# Autodesk Inventor assembly: StraightMF_DSS
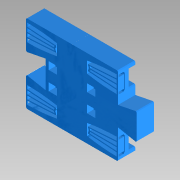
[picture p0: Inventor's stored thumbnail of the model, 180x180]
Saved by Autodesk Inventor 2021 (Build 250183000, 183)
## iProperties
Created: 2021-03-01
Part Number: StraightMF_DSS
Document SubType Name: Assembly
Designer: kumagai
Author: kumagai
## Documents named in this file (11)
- X:\Develop\CAD\PlaRails\StraightRail\StraightRail_i.iam
- X:\Develop\CAD\PlaRails\RailJointMale.ipt
- X:\Develop\CAD\PlaRails\RailJointFemale.ipt
- X:\Develop\CAD\PlaRails\GlobalParameter.ipt
- StraightFF26.iam
- StraightFF60.iam
- StraightMF134.iam
- StraightMF215.iam
- StraightMF_DSS.iam
- StraightMM26.iam
- StraightMM60.iam
## Components (4 placed, 4 different names)
1. M1 — フラッシュ:1, フラッシュ:3, フラッシュ:4
2. M2 — フラッシュ:2, メイト:1, メイト:2
3. F1 — フラッシュ:5, メイト:3, メイト:4
4. F2 — フラッシュ:6, フラッシュ:7, フラッシュ:8
## Relationships (12: Flush 8, Mate 4)
- フラッシュ:1 [Flush]: M1
- フラッシュ:2 [Flush]: M2
- フラッシュ:3 [Flush] (-7.264 mm): M1
- メイト:1 [Mate]: M2
- フラッシュ:4 [Flush]: M1
- メイト:2 [Mate]: M2
- フラッシュ:5 [Flush]: F1
- フラッシュ:6 [Flush]: F2
- フラッシュ:7 [Flush] (-7.264 mm): F2
- フラッシュ:8 [Flush]: F2
- メイト:3 [Mate]: F1
- メイト:4 [Mate]: F1
## Named parameters: Length = 44.52796 mm, ConnectorLength = 15 mm, Offset = 7.26398 mm, StraightLength = 215 mm
